# Autodesk Inventor assembly: RhinoTrackRobotV26
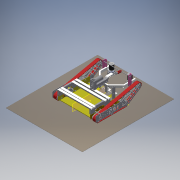
[picture p0: Inventor's stored thumbnail of the model, 180x180]
Saved by Autodesk Inventor 2017 SP1 (Build 210196100, 196)
## iProperties
Created: 2016-02-10
Part Number: RhinoTrackRobotV26
Document SubType Name: Assembly
Designer: steele
Author: steele
## Documents named in this file (11)
- D:\snobotics\CAD-Development\robSteele\SnoBotics2016\2016-08-05-TiltWithVex\RhinoTrackRobotV26.iam
- D:\snobotics\CAD-Development\robSteele\SnoBotics2016\RhinoTrackDriveModule\am-3322+RhinoTrackDriveModule.iam
- D:\snobotics\CAD-Development\robSteele\SnoBotics2016\RhinoBottomFloorOptions\SheetBottomFloorV01.ipt
- D:\snobotics\CAD-Development\robSteele\SnoBotics2016\RhinoBottomFloorOptions\Floor.ipt
- D:\snobotics\CAD-Development\robSteele\SnoBotics2016\DraftOfBoulder.ipt
- D:\snobotics\CAD-Development\robSteele\SnoBotics2016\RhinoTrackDriveModule\am-3322+RhinoTrackDriveModule_MIR15.iam
- D:\snobotics\CAD-Development\robSteele\SnoBotics2016\2016-02-12-RhinoSheetMetalStartOfLift\RailSlideLeftSide.ipt
- D:\snobotics\CAD-Development\robSteele\SnoBotics2016\2016-02-12-RhinoSheetMetalStartOfLift\RailSlideLeftSide_MIR.ipt
- D:\snobotics\CAD-Development\robSteele\SnoBotics2016\2016-02-12-RhinoSheetMetalStartOfLift\3_4x1_1_2_alumTubing.ipt
- D:\snobotics\CAD-Development\robSteele\SnoBotics2016\RobotVolume\RhinoV19MaxVolume.ipt
- D:\snobotics\CAD-Development\robSteele\SnoBotics2016\2016-05-05-ShooterPrototype\ConnectionToDart.iam
## Components (13 placed, 10 different names)
1. am-3322+RhinoTrackDriveModule:1 [sub-assembly] — Mate:1, Flush:1, Flush:2, Mate:4, Mate:37, Flush:9, Mate:38
2. SheetBottomFloorV01:1 — Mate:1, Flush:1, Flush:2, Mate:2, Mate:3, Flush:6, Flush:8, Mate:49, Mate:51, Mate:52, Flush:18
3. Floor:1 — Mate:2, Mate:3, Mate:4, Flush:7, Mate:5, Mate:50
4. DraftOfBoulder:1 — Flush:6, Flush:7, Mate:5
5. am-3322+RhinoTrackDriveModule_MIR15:1 [sub-assembly]
6. RailSlideLeftSide:1 — Mate:37, Flush:9, Mate:38, Mate:39, Flush:10, Flush:11, Mate:40, Flush:12, Mate:41, Mate:42, Flush:13, Mate:43, Mate:44, Flush:14, Mate:45
7. RailSlideLeftSide_MIR:1
8. 3_4x1_1_2_alumTubing:1 — Mate:39, Flush:10, Flush:11
9. 3_4x1_1_2_alumTubing:2 — Mate:40, Flush:12, Mate:41
10. 3_4x1_1_2_alumTubing:3 — Mate:42, Flush:13, Mate:43
11. 3_4x1_1_2_alumTubing:4 — Mate:44, Flush:14, Mate:45
12. RhinoV19MaxVolume:1 — Mate:49, Mate:50
13. ConnectionToDart:1 [sub-assembly] — Mate:51, Mate:52, Flush:18
## Relationships (30: Mate 18, Flush 12)
- Mate:1: am-3322+RhinoTrackDriveModule:1 ↔ SheetBottomFloorV01:1
- Flush:1: am-3322+RhinoTrackDriveModule:1 ↔ SheetBottomFloorV01:1
- Flush:2: am-3322+RhinoTrackDriveModule:1 ↔ SheetBottomFloorV01:1
- Mate:2: SheetBottomFloorV01:1 ↔ Floor:1
- Mate:3: SheetBottomFloorV01:1 ↔ Floor:1
- Mate:4 (0.889 mm): am-3322+RhinoTrackDriveModule:1 ↔ Floor:1
- Flush:6: SheetBottomFloorV01:1 ↔ DraftOfBoulder:1
- Flush:7 (127 mm): Floor:1 ↔ DraftOfBoulder:1
- Mate:5 (-381 mm): Floor:1 ↔ DraftOfBoulder:1
- Flush:8: SheetBottomFloorV01:1
- Mate:37: am-3322+RhinoTrackDriveModule:1 ↔ RailSlideLeftSide:1
- Flush:9: am-3322+RhinoTrackDriveModule:1 ↔ RailSlideLeftSide:1
- Mate:38: am-3322+RhinoTrackDriveModule:1 ↔ RailSlideLeftSide:1
- Mate:39: RailSlideLeftSide:1 ↔ 3_4x1_1_2_alumTubing:1
- Flush:10: RailSlideLeftSide:1 ↔ 3_4x1_1_2_alumTubing:1
- Flush:11: RailSlideLeftSide:1 ↔ 3_4x1_1_2_alumTubing:1
- Mate:40: RailSlideLeftSide:1 ↔ 3_4x1_1_2_alumTubing:2
- Flush:12: RailSlideLeftSide:1 ↔ 3_4x1_1_2_alumTubing:2
- Mate:41: RailSlideLeftSide:1 ↔ 3_4x1_1_2_alumTubing:2
- Mate:42: RailSlideLeftSide:1 ↔ 3_4x1_1_2_alumTubing:3
- Flush:13: RailSlideLeftSide:1 ↔ 3_4x1_1_2_alumTubing:3
- Mate:43: RailSlideLeftSide:1 ↔ 3_4x1_1_2_alumTubing:3
- Mate:44: RailSlideLeftSide:1 ↔ 3_4x1_1_2_alumTubing:4
- Flush:14: RailSlideLeftSide:1 ↔ 3_4x1_1_2_alumTubing:4
- Mate:45: RailSlideLeftSide:1 ↔ 3_4x1_1_2_alumTubing:4
- Mate:49: SheetBottomFloorV01:1 ↔ RhinoV19MaxVolume:1
- Mate:50: Floor:1 ↔ RhinoV19MaxVolume:1
- Mate:51: SheetBottomFloorV01:1 ↔ ConnectionToDart:1
- Mate:52 (31.75 mm): SheetBottomFloorV01:1 ↔ ConnectionToDart:1
- Flush:18 (-436.9562 mm): SheetBottomFloorV01:1 ↔ ConnectionToDart:1
## Named parameters: OffsetBetweenFloorAndLeftTred = 0.889 mm
